# Autodesk Inventor assembly: Microwave Detection Region
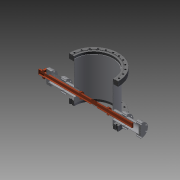
[picture p0: Inventor's stored thumbnail of the model, 180x180]
Saved by Autodesk Inventor 2014 (Build 180170000, 170)
## iProperties
Created: 2014-05-15
Part Number: Microwave Detection Region
Document SubType Name: Assembly
Designer: ijs09
Author: ijs09
## Documents named in this file (14)
- D:\Inventor\CCM CAD Files\CADFiles\Microwave Detection Region\Microwave Detection Region.iam
- D:\Inventor\CCM CAD Files\CADFiles\Microwave Detection Region\Waveguide.ipt
- D:\Inventor\CCM CAD Files\CADFiles\Microwave Detection Region\WG17FlangeCutDown.ipt
- D:\Inventor\CCM CAD Files\CADFiles\Microwave Detection Region\Waveguide Terminator.ipt
- D:\Inventor\CCM CAD Files\CADFiles\Microwave Detection Region\Waveguide Feedthrough.ipt
- D:\Inventor\CCM CAD Files\CADFiles\Microwave Detection Region\WG17FLANGE.ipt
- D:\Inventor\CCM CAD Files\CADFiles\Microwave Detection Region\Coaxial Feed.ipt
- D:\Inventor\CCM CAD Files\CADFiles\Microwave Detection Region\Detection Region Vacuum Collar.ipt
- D:\Inventor\CCM CAD Files\CADFiles\Microwave Detection Region\DN200CF.ipt
- D:\Inventor\CCM CAD Files\CADFiles\Microwave Detection Region\DN35CF Counter Bored.ipt
- D:\Inventor\CCM CAD Files\CADFiles\Microwave Detection Region\Bellows.ipt
- D:\Inventor\CCM CAD Files\CADFiles\Microwave Detection Region\Waveguide Terminator Nipple.ipt
- D:\Inventor\CCM CAD Files\CADFiles\Microwave Detection Region\DN35CF Blank.ipt
- D:\Inventor\CCM CAD Files\CADFiles\Microwave Detection Region\MellesGriot01MCG023.ipt
## Components (22 placed, 13 different names)
1. Waveguide:1 — Flush:1, Flush:2, Mate:3, Mate:4, Mate:5, Mate:6, Mate:11, Mate:12, Mate:13, Mate:16, Mate:17
2. WG17FlangeCutDown:1 — Flush:1, Mate:5, Mate:6, Mate:7
3. WG17FlangeCutDown:2 — Flush:2, Mate:3, Mate:4
4. Waveguide Terminator:1 — Mate:7, Flush:3, Mate:8, Mate:9, Mate:11, Mate:12
5. WG17FlangeCutDown:3 — Flush:3, Mate:8, Mate:9
6. Waveguide Feedthrough:1 — Mate:13, Flush:4, Mate:14, Mate:15, Mate:16, Mate:17, Flush:5, Mate:18, Mate:19, Mate:39, Mate:40
7. WG17FlangeCutDown:4 — Flush:4, Mate:14, Mate:15
8. WG17FLANGE:1 — Flush:5, Mate:18, Mate:19, Mate:20, Mate:22, Mate:23
9. Coaxial Feed:1 — Mate:20, Mate:22, Mate:23
10. Detection Region Vacuum Collar:1 — Mate:24, Mate:25, Mate:26, Mate:27, Mate:28, Mate:29, Mate:30, Mate:31, Mate:37, Mate:46
11. DN200CF:1 — Mate:24, Mate:25
12. DN200CF:2 — Mate:26, Mate:27
13. DN35CF Counter Bored:1 — Mate:28, Mate:29, Mate:45
14. DN35CF Counter Bored:2 — Mate:30, Mate:31, Mate:36, Mate:38
15. Bellows:1 — Mate:32, Mate:33, Mate:34, Mate:35, Mate:37, Mate:40
16. DN35CF Counter Bored:3 — Mate:32, Mate:33, Mate:36, Mate:38
17. DN35CF Counter Bored:4 — Mate:34, Mate:35, Mate:39
18. Waveguide Terminator Nipple:1 — Mate:41, Mate:42, Mate:46, Mate:47, Mate:48, Mate:50
19. DN35CF Counter Bored:6 — Mate:41, Mate:42, Mate:45
20. DN35CF Counter Bored:7 — Mate:47, Mate:48, Mate:49
21. DN35CF Blank:1 — Mate:49, Mate:50
22. MellesGriot01MCG023:1
## Relationships (49: Mate 44, Flush 5)
- Flush:1: Waveguide:1 ↔ WG17FlangeCutDown:1
- Flush:2: Waveguide:1 ↔ WG17FlangeCutDown:2
- Mate:3: Waveguide:1 ↔ WG17FlangeCutDown:2
- Mate:4: Waveguide:1 ↔ WG17FlangeCutDown:2
- Mate:5: Waveguide:1 ↔ WG17FlangeCutDown:1
- Mate:6: Waveguide:1 ↔ WG17FlangeCutDown:1
- Mate:7: WG17FlangeCutDown:1 ↔ Waveguide Terminator:1
- Flush:3: Waveguide Terminator:1 ↔ WG17FlangeCutDown:3
- Mate:8: Waveguide Terminator:1 ↔ WG17FlangeCutDown:3
- Mate:9: Waveguide Terminator:1 ↔ WG17FlangeCutDown:3
- Mate:11: Waveguide:1 ↔ Waveguide Terminator:1
- Mate:12: Waveguide:1 ↔ Waveguide Terminator:1
- Mate:13: Waveguide:1 ↔ Waveguide Feedthrough:1
- Flush:4: Waveguide Feedthrough:1 ↔ WG17FlangeCutDown:4
- Mate:14: Waveguide Feedthrough:1 ↔ WG17FlangeCutDown:4
- Mate:15: Waveguide Feedthrough:1 ↔ WG17FlangeCutDown:4
- Mate:16: Waveguide:1 ↔ Waveguide Feedthrough:1
- Mate:17: Waveguide:1 ↔ Waveguide Feedthrough:1
- Flush:5: Waveguide Feedthrough:1 ↔ WG17FLANGE:1
- Mate:18: Waveguide Feedthrough:1 ↔ WG17FLANGE:1
- Mate:19: Waveguide Feedthrough:1 ↔ WG17FLANGE:1
- Mate:20: WG17FLANGE:1 ↔ Coaxial Feed:1
- Mate:22: WG17FLANGE:1 ↔ Coaxial Feed:1
- Mate:23: WG17FLANGE:1 ↔ Coaxial Feed:1
- Mate:24: Detection Region Vacuum Collar:1 ↔ DN200CF:1
- Mate:25: Detection Region Vacuum Collar:1 ↔ DN200CF:1
- Mate:26: Detection Region Vacuum Collar:1 ↔ DN200CF:2
- Mate:27: Detection Region Vacuum Collar:1 ↔ DN200CF:2
- Mate:28: Detection Region Vacuum Collar:1 ↔ DN35CF Counter Bored:1
- Mate:29: Detection Region Vacuum Collar:1 ↔ DN35CF Counter Bored:1
- Mate:30: Detection Region Vacuum Collar:1 ↔ DN35CF Counter Bored:2
- Mate:31: Detection Region Vacuum Collar:1 ↔ DN35CF Counter Bored:2
- Mate:32: Bellows:1 ↔ DN35CF Counter Bored:3
- Mate:33: Bellows:1 ↔ DN35CF Counter Bored:3
- Mate:34: Bellows:1 ↔ DN35CF Counter Bored:4
- Mate:35: Bellows:1 ↔ DN35CF Counter Bored:4
- Mate:36: DN35CF Counter Bored:2 ↔ DN35CF Counter Bored:3
- Mate:37: Detection Region Vacuum Collar:1 ↔ Bellows:1
- Mate:38: DN35CF Counter Bored:2 ↔ DN35CF Counter Bored:3
- Mate:39: Waveguide Feedthrough:1 ↔ DN35CF Counter Bored:4
- Mate:40: Waveguide Feedthrough:1 ↔ Bellows:1
- Mate:41: Waveguide Terminator Nipple:1 ↔ DN35CF Counter Bored:6
- Mate:42: Waveguide Terminator Nipple:1 ↔ DN35CF Counter Bored:6
- Mate:45: DN35CF Counter Bored:1 ↔ DN35CF Counter Bored:6
- Mate:46: Detection Region Vacuum Collar:1 ↔ Waveguide Terminator Nipple:1
- Mate:47: Waveguide Terminator Nipple:1 ↔ DN35CF Counter Bored:7
- Mate:48: Waveguide Terminator Nipple:1 ↔ DN35CF Counter Bored:7
- Mate:49: DN35CF Counter Bored:7 ↔ DN35CF Blank:1
- Mate:50: Waveguide Terminator Nipple:1 ↔ DN35CF Blank:1
